# Autodesk Inventor assembly: Lidarbase
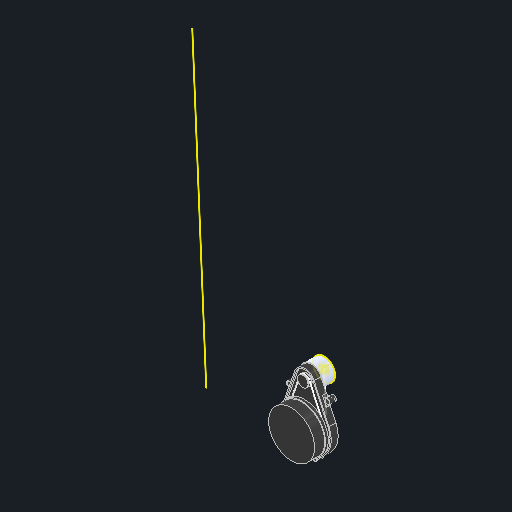
[picture p0: Inventor's stored thumbnail of the model, 512x512]
Saved by Autodesk Inventor 2026.1 (Build 301233020, 233B)
## iProperties
Created: 2025-12-01
Part Number: Lidarbase
Document SubType Name: Assembly
Designer: jaewook
Author: jaewook
## Documents named in this file (3)
- C:\Users\kjh19\Documents\Inventor\project\final\Lidarbase.iam
- C:\Users\kjh19\Documents\Inventor\project\final\Lidar.ipt
- C:\Users\kjh19\Downloads\ydlidar-x4pro-1.snapshot.6\LIDAR X4 PRO.ipt
## Components (2 placed, 2 different names)
1. Lidar_base:1 — 메이트:1
2. LIDAR X4 PRO:1 — 메이트:1
## Relationships (1: Mate 1)
- 메이트:1 [Mate]: Lidar_base:1 ↔ LIDAR X4 PRO:1
